# Autodesk Inventor assembly: Assembly2
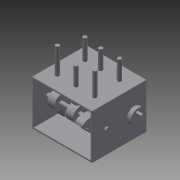
[picture p0: Inventor's stored thumbnail of the model, 180x180]
Saved by Autodesk Inventor 2014 (Build 180170000, 170)
## iProperties
Created: 2014-05-19
Part Number: Assembly2
Document SubType Name: Assembly
Designer: jyesowitz
Author: jyesowitz
## Documents named in this file (8)
- C:\Users\jyesowitz\Documents\GitHub\FinalProjectFirst\Assembly2.iam
- C:\Users\jyesowitz\Documents\GitHub\FinalProjectFirst\cam 1.ipt
- C:\Users\jyesowitz\Documents\GitHub\FinalProjectFirst\cam 2.ipt
- C:\Users\jyesowitz\Documents\GitHub\FinalProjectFirst\cam 3.ipt
- C:\Users\jyesowitz\Documents\GitHub\FinalProjectFirst\rod.ipt
- C:\Users\jyesowitz\Documents\GitHub\FinalProjectFirst\Box Base.ipt
- C:\Users\jyesowitz\Documents\GitHub\FinalProjectFirst\crank.ipt
- C:\Users\jyesowitz\Documents\GitHub\FinalProjectFirst\moving ball thing.ipt
## Components (17 placed, 7 different names)
1. cam 1:1 — Insert:3, Flush:6
2. cam 2:1 — Insert:1, Flush:5
3. cam 3:1 — Insert:2, Flush:7
4. rod:1 — Insert:1, Insert:2, Insert:3, Mate:12, Mate:13, Insert:9
5. cam 1:2 — Insert:5, Flush:9
6. cam 2:2 — Insert:6, Flush:8
7. cam 3:2 — Insert:4, Flush:10
8. rod:2 — Insert:4, Insert:5, Insert:6, Mate:10, Mate:11, Insert:10
9. Box Base:1 — Mate:1, Mate:2, Angle:2, Angle:3, Angle:4, Angle:5, Angle:6, Angle:7, Insert:9, Insert:10, Mate:14, Mate:15, Mate:16, Mate:17, Mate:18, Mate:19
10. crank:1 — Mate:12, Mate:13
11. crank:2 — Mate:10, Mate:11
12. moving ball thing:1 — Angle:2, Mate:14
13. moving ball thing:2 — Angle:6, Mate:19
14. moving ball thing:3 — Angle:3, Mate:15
15. moving ball thing:4 — Angle:7, Mate:16
16. moving ball thing:5 — Angle:5, Mate:17
17. moving ball thing:6 — Angle:4, Mate:18
## Relationships (32: Mate 12, Insert 8, Angle 6, Flush 6)
- Insert:1 (38.1 mm): cam 2:1 ↔ rod:1
- Insert:2 (29.21 mm): cam 3:1 ↔ rod:1
- Insert:3 (101.6 mm): cam 1:1 ↔ rod:1
- Insert:4 (31.75 mm): cam 3:2 ↔ rod:2
- Insert:5 (25.4 mm): cam 1:2 ↔ rod:2
- Insert:6 (95.25 mm): cam 2:2 ↔ rod:2
- Mate:1: Box Base:1
- Mate:2: Box Base:1
- Angle:2 (0 deg): Box Base:1 ↔ moving ball thing:1
- Angle:3 (0 deg): Box Base:1 ↔ moving ball thing:3
- Angle:4 (0 deg): Box Base:1 ↔ moving ball thing:6
- Angle:5 (0 deg): Box Base:1 ↔ moving ball thing:5
- Angle:6 (0 deg): Box Base:1 ↔ moving ball thing:2
- Angle:7 (0 deg): Box Base:1 ↔ moving ball thing:4
- Mate:10: rod:2 ↔ crank:2
- Mate:11: rod:2 ↔ crank:2
- Mate:12: rod:1 ↔ crank:1
- Mate:13: rod:1 ↔ crank:1
- Insert:9 (-6.35 mm): rod:1 ↔ Box Base:1
- Insert:10 (-6.35 mm): rod:2 ↔ Box Base:1
- Flush:5 (-12.7 mm): cam 2:1
- Flush:6 (-12.7 mm): cam 1:1
- Flush:7 (-12.7 mm): cam 3:1
- Flush:8 (-12.7 mm): cam 2:2
- Flush:9 (-12.7 mm): cam 1:2
- Flush:10 (-12.7 mm): cam 3:2
- Mate:14: Box Base:1 ↔ moving ball thing:1
- Mate:15: Box Base:1 ↔ moving ball thing:3
- Mate:16: Box Base:1 ↔ moving ball thing:4
- Mate:17: Box Base:1 ↔ moving ball thing:5
- Mate:18: Box Base:1 ↔ moving ball thing:6
- Mate:19: Box Base:1 ↔ moving ball thing:2
